# Autodesk Inventor assembly: move_straight
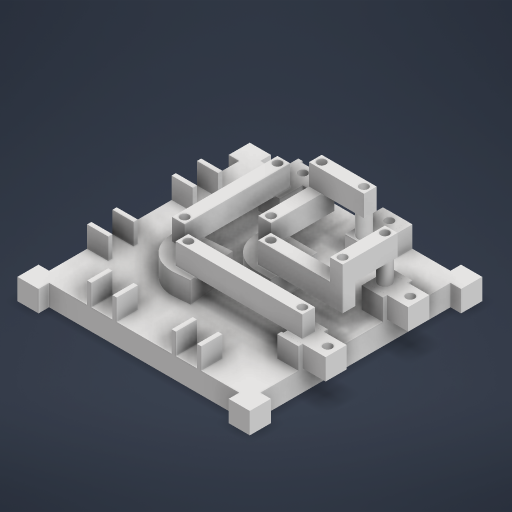
[picture p0: Inventor's stored thumbnail of the model, 512x512]
Saved by Autodesk Inventor 2024.3 (Build 283343000, 343)
## iProperties
Created: 2024-09-29
Part Number: move_straight
Document SubType Name: Assembly
Designer: sam
Author: sam
## Documents named in this file (10)
- N:\Cad\computer\gates\move_right.iam
- N:\Cad\computer\gates\base.ipt
- N:\Cad\computer\gates\block.ipt
- N:\Cad\computer\gates\bellcrank.ipt
- N:\Cad\computer\gates\arm_bellcrank.ipt
- N:\Cad\computer\gates\arm_bellcrank_small.ipt
- N:\Cad\computer\gates\larm_bellcrank.ipt
- N:\Cad\computer\gates\larm_bellcrank_small.ipt
- N:\Cad\computer\gates\spacer_small.ipt
- N:\Cad\computer\gates\bar_bellcrank.ipt
## Components (15 placed, 9 different names)
1. base:1 — Mate:2, Mate:4, Mate:5, Mate:6, Mate:7, Mate:8, Mate:9, Mate:10, Mate:11, Mate:12, Mate:23, Mate:24
2. block:1 — Mate:2, Mate:6, Mate:38, Mate:39, Flush:1, Flush:3
3. block:4 — Mate:4, Mate:5, Mate:15, Mate:17
4. block:5 — Mate:8, Mate:9, Mate:20, Mate:21
5. block:6 — Mate:7, Mate:10, Mate:40, Mate:41, Flush:2
6. bellcrank:2 — Mate:11, Mate:12, Mate:19, Mate:22
7. arm_bellcrank:1 — Mate:15, Mate:17, Mate:19
8. arm_bellcrank_small:1 — Mate:20, Mate:21, Mate:22
9. bellcrank:3 — Mate:23, Mate:24, Mate:34, Mate:35, Mate:36, Mate:37
10. larm_bellcrank:1 — Mate:34, Mate:35, Mate:44
11. larm_bellcrank_small:1 — Mate:36, Mate:37, Mate:47, Mate:48
12. spacer_small:1 — Mate:38, Mate:39, Mate:42, Mate:43
13. spacer_small:2 — Mate:40, Mate:41, Mate:45, Mate:46
14. bar_bellcrank:1 — Mate:42, Flush:1, Mate:43, Mate:44, Flush:3
15. bar_bellcrank:2 — Mate:45, Mate:46, Mate:47, Mate:48, Flush:2
## Relationships (36: Mate 33, Flush 3)
- Mate:2: base:1 ↔ block:1
- Mate:4: base:1 ↔ block:4
- Mate:5: base:1 ↔ block:4
- Mate:6: base:1 ↔ block:1
- Mate:7: base:1 ↔ block:6
- Mate:8: base:1 ↔ block:5
- Mate:9: base:1 ↔ block:5
- Mate:10: base:1 ↔ block:6
- Mate:11: base:1 ↔ bellcrank:2
- Mate:12: base:1 ↔ bellcrank:2
- Mate:15: block:4 ↔ arm_bellcrank:1
- Mate:17: block:4 ↔ arm_bellcrank:1
- Mate:19: bellcrank:2 ↔ arm_bellcrank:1
- Mate:20: block:5 ↔ arm_bellcrank_small:1
- Mate:21: block:5 ↔ arm_bellcrank_small:1
- Mate:22: bellcrank:2 ↔ arm_bellcrank_small:1
- Mate:23: base:1 ↔ bellcrank:3
- Mate:24: base:1 ↔ bellcrank:3
- Mate:34: bellcrank:3 ↔ larm_bellcrank:1
- Mate:35: bellcrank:3 ↔ larm_bellcrank:1
- Mate:36: bellcrank:3 ↔ larm_bellcrank_small:1
- Mate:37: bellcrank:3 ↔ larm_bellcrank_small:1
- Mate:38: block:1 ↔ spacer_small:1
- Mate:39: block:1 ↔ spacer_small:1
- Mate:40: block:6 ↔ spacer_small:2
- Mate:41: block:6 ↔ spacer_small:2
- Mate:42: spacer_small:1 ↔ bar_bellcrank:1
- Flush:1 (1 mm): block:1 ↔ bar_bellcrank:1
- Mate:43: spacer_small:1 ↔ bar_bellcrank:1
- Mate:44: larm_bellcrank:1 ↔ bar_bellcrank:1
- Mate:45: spacer_small:2 ↔ bar_bellcrank:2
- Mate:46: spacer_small:2 ↔ bar_bellcrank:2
- Mate:47: larm_bellcrank_small:1 ↔ bar_bellcrank:2
- Mate:48: larm_bellcrank_small:1 ↔ bar_bellcrank:2
- Flush:2 (1 mm): block:6 ↔ bar_bellcrank:2
- Flush:3 (1 mm): block:1 ↔ bar_bellcrank:1
